# Autodesk Inventor assembly: InterfaceBlock-OutPCB-Connectors
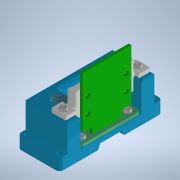
[picture p0: Inventor's stored thumbnail of the model, 180x180]
Saved by Autodesk Inventor 2021 (Build 250183000, 183)
## iProperties
Created: 2020-04-07
Part Number: InterfaceBlock-OutPCB-Connectors
Document SubType Name: Assembly
Designer: jgray
Author: jgray
## Documents named in this file (9)
- M:\Printed Electronics\Gas Sensors\Prototypes\Prototype II -Cartridge Reader V3\InterfaceBlock-OutPCB-Connectors.iam
- M:\Printed Electronics\Gas Sensors\Prototypes\Prototype II -Cartridge Reader V3\RS 278-534 M3 fixing Dia4FixHole.ipt
- M:\Printed Electronics\Gas Sensors\Prototypes\Prototype II -Cartridge Reader V3\Out-PCB plus Connectors.iam
- M:\Printed Electronics\Gas Sensors\Prototypes\Prototype II -Cartridge Reader V3\ANSI B18.3.4M - M3 x 0.5 x 8(1).ipt
- M:\Printed Electronics\Gas Sensors\Prototypes\Prototype II -Cartridge Reader V3\IS 5371 - B3.2.ipt
- M:\Printed Electronics\Gas Sensors\Prototypes\Prototype II -Cartridge Reader V3\ANSI B18.3.4M - M3 x 0.5 x 6(1).ipt
- M:\Printed Electronics\Gas Sensors\Prototypes\Prototype II -Cartridge Reader V3\PCB cross support bracket.ipt
- M:\Printed Electronics\Gas Sensors\Prototypes\Prototype II -Cartridge Reader V3\Extension Board Assembly.iam
- M:\Printed Electronics\Gas Sensors\Prototypes\Prototype II -Cartridge Reader V3\Box Support block Mach.ipt
## Components (23 placed, 8 different names)
1. Box Support block Mach:1 — Mate:1, Mate:2, Mate:3, Mate:4, Flush:4, Mate:5, Mate:24, Mate:25, Flush:5, Flush:6, Mate:26, Mate:27, Angle:3, Angle:4
2. RS 278-534 M3 fixing Dia4FixHole:1 — Mate:4, Flush:1, Flush:2, Flush:3, Flush:4
3. RS 278-534 M3 fixing Dia4FixHole:2 — Mate:1, Flush:2
4. RS 278-534 M3 fixing Dia4FixHole:3 — Mate:3, Flush:3, Mate:7
5. RS 278-534 M3 fixing Dia4FixHole:4 — Mate:2, Flush:1, Mate:6
6. Out-PCB plus Connectors:1 [sub-assembly] — Mate:5, Mate:6, Mate:7, Mate:16, Mate:17, Mate:18, Mate:19, Mate:20, Mate:21, Mate:22, Mate:23, Mate:46
7. Forged Hexagon Socket Button Head Cap Screw - Metric M3 x 0.5 x 8:1 — Mate:11, Mate:15, Mate:22
8. Forged Hexagon Socket Button Head Cap Screw - Metric M3 x 0.5 x 6:1 — Mate:10, Mate:14, Mate:21
9. Forged Hexagon Socket Button Head Cap Screw - Metric M3 x 0.5 x 6:2 — Mate:8, Mate:12, Mate:23
10. Forged Hexagon Socket Button Head Cap Screw - Metric M3 x 0.5 x 6:3 — Mate:9, Mate:13, Mate:20
11. IS 5371 B B3.2:1 — Mate:8, Mate:12, Mate:16
12. IS 5371 B B3.2:2 — Mate:9, Mate:13, Mate:17
13. IS 5371 B B3.2:3 — Mate:11, Mate:15, Mate:19
14. IS 5371 B B3.2:4 — Mate:10, Mate:14, Mate:18
15. RS 278-534 M3 fixing Dia4FixHole:5 — Mate:24, Flush:5, Mate:30, Mate:31, Mate:38
16. RS 278-534 M3 fixing Dia4FixHole:6 — Mate:25, Flush:6, Mate:28, Mate:29, Mate:39
17. PCB cross support bracket:1 — Mate:26, Mate:28, Mate:29, Angle:1, Mate:36, Flush:9
18. PCB cross support bracket:2 — Mate:27, Mate:30, Mate:31, Angle:1, Mate:37, Flush:9, Angle:4, Mate:47
19. Forged Hexagon Socket Button Head Cap Screw - Metric M3 x 0.5 x 8:2 — Mate:33, Mate:34, Mate:39
20. Forged Hexagon Socket Button Head Cap Screw - Metric M3 x 0.5 x 8:3 — Mate:32, Mate:35, Mate:38
21. IS 5371 B B3.2:5 — Mate:32, Mate:35, Mate:37
22. IS 5371 B B3.2:6 — Mate:33, Mate:34, Mate:36
23. Extension Board Assembly:1 [sub-assembly] — Mate:46, Mate:47
## Relationships (51: Mate 41, Flush 7, Angle 3)
- Mate:1: Box Support block Mach:1 ↔ RS 278-534 M3 fixing Dia4FixHole:2
- Mate:2: Box Support block Mach:1 ↔ RS 278-534 M3 fixing Dia4FixHole:4
- Mate:3: Box Support block Mach:1 ↔ RS 278-534 M3 fixing Dia4FixHole:3
- Mate:4: Box Support block Mach:1 ↔ RS 278-534 M3 fixing Dia4FixHole:1
- Flush:1: RS 278-534 M3 fixing Dia4FixHole:1 ↔ RS 278-534 M3 fixing Dia4FixHole:4
- Flush:2: RS 278-534 M3 fixing Dia4FixHole:1 ↔ RS 278-534 M3 fixing Dia4FixHole:2
- Flush:3: RS 278-534 M3 fixing Dia4FixHole:1 ↔ RS 278-534 M3 fixing Dia4FixHole:3
- Flush:4: Box Support block Mach:1 ↔ RS 278-534 M3 fixing Dia4FixHole:1
- Mate:5: Box Support block Mach:1 ↔ Out-PCB plus Connectors:1
- Mate:6: RS 278-534 M3 fixing Dia4FixHole:4 ↔ Out-PCB plus Connectors:1
- Mate:7: RS 278-534 M3 fixing Dia4FixHole:3 ↔ Out-PCB plus Connectors:1
- Mate:8: Forged Hexagon Socket Button Head Cap Screw - Metric M3 x 0.5 x 6:2 ↔ IS 5371 B B3.2:1
- Mate:9: Forged Hexagon Socket Button Head Cap Screw - Metric M3 x 0.5 x 6:3 ↔ IS 5371 B B3.2:2
- Mate:10: Forged Hexagon Socket Button Head Cap Screw - Metric M3 x 0.5 x 6:1 ↔ IS 5371 B B3.2:4
- Mate:11: Forged Hexagon Socket Button Head Cap Screw - Metric M3 x 0.5 x 8:1 ↔ IS 5371 B B3.2:3
- Mate:12: Forged Hexagon Socket Button Head Cap Screw - Metric M3 x 0.5 x 6:2 ↔ IS 5371 B B3.2:1
- Mate:13: Forged Hexagon Socket Button Head Cap Screw - Metric M3 x 0.5 x 6:3 ↔ IS 5371 B B3.2:2
- Mate:14: Forged Hexagon Socket Button Head Cap Screw - Metric M3 x 0.5 x 6:1 ↔ IS 5371 B B3.2:4
- Mate:15: Forged Hexagon Socket Button Head Cap Screw - Metric M3 x 0.5 x 8:1 ↔ IS 5371 B B3.2:3
- Mate:16: Out-PCB plus Connectors:1 ↔ IS 5371 B B3.2:1
- Mate:17: Out-PCB plus Connectors:1 ↔ IS 5371 B B3.2:2
- Mate:18: Out-PCB plus Connectors:1 ↔ IS 5371 B B3.2:4
- Mate:19: Out-PCB plus Connectors:1 ↔ IS 5371 B B3.2:3
- Mate:20: Out-PCB plus Connectors:1 ↔ Forged Hexagon Socket Button Head Cap Screw - Metric M3 x 0.5 x 6:3
- Mate:21: Out-PCB plus Connectors:1 ↔ Forged Hexagon Socket Button Head Cap Screw - Metric M3 x 0.5 x 6:1
- Mate:22: Out-PCB plus Connectors:1 ↔ Forged Hexagon Socket Button Head Cap Screw - Metric M3 x 0.5 x 8:1
- Mate:23: Out-PCB plus Connectors:1 ↔ Forged Hexagon Socket Button Head Cap Screw - Metric M3 x 0.5 x 6:2
- Mate:24: Box Support block Mach:1 ↔ RS 278-534 M3 fixing Dia4FixHole:5
- Mate:25: Box Support block Mach:1 ↔ RS 278-534 M3 fixing Dia4FixHole:6
- Flush:5: Box Support block Mach:1 ↔ RS 278-534 M3 fixing Dia4FixHole:5
- Flush:6: Box Support block Mach:1 ↔ RS 278-534 M3 fixing Dia4FixHole:6
- Mate:26: Box Support block Mach:1 ↔ PCB cross support bracket:1
- Mate:27: Box Support block Mach:1 ↔ PCB cross support bracket:2
- Mate:28 (0.5 mm): RS 278-534 M3 fixing Dia4FixHole:6 ↔ PCB cross support bracket:1
- Mate:29 (0.5 mm): RS 278-534 M3 fixing Dia4FixHole:6 ↔ PCB cross support bracket:1
- Mate:30 (-0.5 mm): RS 278-534 M3 fixing Dia4FixHole:5 ↔ PCB cross support bracket:2
- Mate:31 (0.5 mm): RS 278-534 M3 fixing Dia4FixHole:5 ↔ PCB cross support bracket:2
- Angle:1 (0 deg): PCB cross support bracket:1 ↔ PCB cross support bracket:2
- Mate:32: Forged Hexagon Socket Button Head Cap Screw - Metric M3 x 0.5 x 8:3 ↔ IS 5371 B B3.2:5
- Mate:33: Forged Hexagon Socket Button Head Cap Screw - Metric M3 x 0.5 x 8:2 ↔ IS 5371 B B3.2:6
- Mate:34: Forged Hexagon Socket Button Head Cap Screw - Metric M3 x 0.5 x 8:2 ↔ IS 5371 B B3.2:6
- Mate:35: Forged Hexagon Socket Button Head Cap Screw - Metric M3 x 0.5 x 8:3 ↔ IS 5371 B B3.2:5
- Mate:36: PCB cross support bracket:1 ↔ IS 5371 B B3.2:6
- Mate:37: PCB cross support bracket:2 ↔ IS 5371 B B3.2:5
- Mate:38: RS 278-534 M3 fixing Dia4FixHole:5 ↔ Forged Hexagon Socket Button Head Cap Screw - Metric M3 x 0.5 x 8:3
- Mate:39: RS 278-534 M3 fixing Dia4FixHole:6 ↔ Forged Hexagon Socket Button Head Cap Screw - Metric M3 x 0.5 x 8:2
- Flush:9: PCB cross support bracket:1 ↔ PCB cross support bracket:2
- Angle:3 (0 deg): Box Support block Mach:1
- Angle:4 (0 deg): Box Support block Mach:1 ↔ PCB cross support bracket:2
- Mate:46: Out-PCB plus Connectors:1 ↔ Extension Board Assembly:1
- Mate:47: PCB cross support bracket:2 ↔ Extension Board Assembly:1
